# Autodesk Inventor assembly: Assembly_that_isnt_completly broken
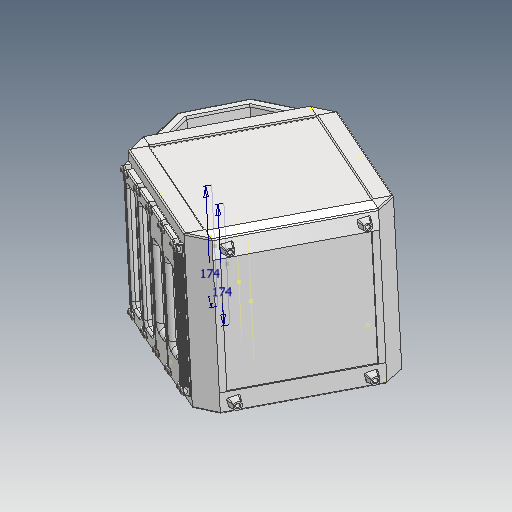
[picture p0: Inventor's stored thumbnail of the model, 512x512]
Saved by Autodesk Inventor 2027 (Build 310192060, 192F)
## iProperties
Created: 2026-07-30
Part Number: Assembly_that_isnt_completly broken
Document SubType Name: Assembly
Designer: prest
Author: prest
## Documents named in this file (14)
- C:\Users\prest\OneDrive\Documents\Projects\Home_Lab_Rack\Assembly_that_isnt_completly broken.iam
- C:\Users\prest\OneDrive\Documents\Projects\Home_Lab_Rack\Strut_Angled.ipt
- C:\Users\prest\OneDrive\Documents\Projects\Home_Lab_Rack\Strut_Horizonal_Bottom.ipt
- C:\Users\prest\OneDrive\Documents\Projects\Home_Lab_Rack\Strut_Horizonal_Top.ipt
- C:\Users\prest\OneDrive\Documents\Projects\Home_Lab_Rack\Strut_Vertical.ipt
- C:\Users\prest\OneDrive\Documents\Projects\Home_Lab_Rack\Panel_Bottom.ipt
- C:\Users\prest\OneDrive\Documents\Projects\Home_Lab_Rack\Panel_Side.ipt
- C:\Users\prest\OneDrive\Documents\Projects\Home_Lab_Rack\MISC\Feet.ipt
- C:\Users\prest\OneDrive\Documents\Projects\Home_Lab_Rack\MISC\Handle.ipt
- C:\Users\prest\OneDrive\Documents\Projects\Home_Lab_Rack\Mounts\router_mount.ipt
- C:\Users\prest\OneDrive\Documents\Projects\Home_Lab_Rack\Mounts\Front_Panel_Breathers.ipt
- C:\Users\prest\OneDrive\Documents\Projects\Home_Lab_Rack\Mounts\mini_PC_mount.ipt
- C:\Users\prest\OneDrive\Documents\Inventor\Content Center Files\R2027\en-US\BS 4168(6)\BS 4168 - M6 x 12(6).ipt
- C:\Users\prest\OneDrive\Documents\Projects\Home_Lab_Rack\Panel_Top.ipt
## Components (62 placed, 13 different names)
1. Strut_Angled:1 — Rigid:5, Rigid:6, Rigid:7, Rotational:32, Rotational:33, Mate:30, Rigid:14
2. Strut_Horizonal_Bottom:1 — Rigid:3, Rigid:5, Rotational:6, Rotational:7
3. Strut_Horizonal_Bottom:2 — Rotational:3, Rotational:4, Rotational:5, Mate:30
4. Strut_Vertical:1 — Rigid:1, Rigid:8, Mate:2, Mate:4, Mate:6, Mate:8, Mate:11, Mate:14, Mate:18, Rigid:11
5. Strut_Angled:2 — Rigid:1, Rigid:3, Rigid:4, Mate:16, Rotational:3
6. Strut_Angled:3 — Rigid:8, Rotational:2, Mate:13, Mate:20, Rotational:36, Rotational:37, Rotational:38, Rotational:39
7. Strut_Vertical:2 — Rigid:4, Mate:1, Mate:3, Mate:5, Mate:7, Mate:9, Mate:10, Mate:12, Mate:15, Mate:17, Rigid:12
8. Strut_Vertical:3 — Rigid:7, Rigid:9
9. Strut_Vertical:4 — Rigid:6
10. Strut_Angled:4 — Rigid:9, Rotational:1, Mate:19, Rotational:34, Rotational:35, Rotational:40, Rotational:41
11. Strut_Horizonal_Top:2 — Rotational:1, Mate:20, Rigid:10
12. Strut_Horizonal_Top:3 — Rotational:2, Mate:19, Mate:21, Mate:22, Rigid:15
13. Feet:1 — Rotational:7
14. router_mount:1 — Mate:1, Mate:2, Mate:3, Rotational:21, Rotational:22, Rotational:24, Rotational:25
15. Front_Panel_Breathers:1 — Mate:13, Mate:14, Mate:15, Rotational:8, Rotational:9
16. mini_PC_mount:1 — Mate:7, Mate:8, Mate:9, Rotational:13, Rotational:15, Rotational:16, Rotational:17
17. router_mount:2 — Mate:4, Mate:5, Mate:6, Rotational:18, Rotational:19, Rotational:20, Rotational:23
18. mini_PC_mount:2 — Mate:10, Mate:11, Mate:12, Rotational:10, Rotational:11, Rotational:12, Rotational:14
19. Front_Panel_Breathers:2 — Mate:16, Mate:17, Mate:18, Rotational:26, Rotational:27
20. Handle:1 — Rigid:10, Rotational:29, Rotational:30
21. Handle:2 — Mate:21, Mate:22, Rotational:28, Rotational:31
22. Feet:2 — Rotational:4
23. Feet:3 — Rotational:5
24. Feet:4 — Rotational:6
25. BS 4168 : Part 6 Hexagon socket countersunk and button head screws - Metric series - Metric M6 x 12:1 — Rotational:32
26. BS 4168 : Part 6 Hexagon socket countersunk and button head screws - Metric series - Metric M6 x 12:2 — Rotational:35
27. BS 4168 : Part 6 Hexagon socket countersunk and button head screws - Metric series - Metric M6 x 12:3 — Rotational:36
28. BS 4168 : Part 6 Hexagon socket countersunk and button head screws - Metric series - Metric M6 x 12:4 — Rotational:37
29. BS 4168 : Part 6 Hexagon socket countersunk and button head screws - Metric series - Metric M6 x 12:5 — Rotational:40
30. BS 4168 : Part 6 Hexagon socket countersunk and button head screws - Metric series - Metric M6 x 12:6 — Rotational:41
31. BS 4168 : Part 6 Hexagon socket countersunk and button head screws - Metric series - Metric M6 x 12:7 — Rotational:9
32. BS 4168 : Part 6 Hexagon socket countersunk and button head screws - Metric series - Metric M6 x 12:8 — Rotational:8
33. BS 4168 : Part 6 Hexagon socket countersunk and button head screws - Metric series - Metric M6 x 12:9 — Rotational:28
34. BS 4168 : Part 6 Hexagon socket countersunk and button head screws - Metric series - Metric M6 x 12:10 — Rotational:34
35. BS 4168 : Part 6 Hexagon socket countersunk and button head screws - Metric series - Metric M6 x 12:11 — Rotational:10
36. BS 4168 : Part 6 Hexagon socket countersunk and button head screws - Metric series - Metric M6 x 12:12 — Rotational:11
37. BS 4168 : Part 6 Hexagon socket countersunk and button head screws - Metric series - Metric M6 x 12:13 — Rotational:12
38. BS 4168 : Part 6 Hexagon socket countersunk and button head screws - Metric series - Metric M6 x 12:14 — Rotational:13
39. BS 4168 : Part 6 Hexagon socket countersunk and button head screws - Metric series - Metric M6 x 12:15 — Rotational:15
40. BS 4168 : Part 6 Hexagon socket countersunk and button head screws - Metric series - Metric M6 x 12:16 — Rotational:14
41. BS 4168 : Part 6 Hexagon socket countersunk and button head screws - Metric series - Metric M6 x 12:17 — Rotational:27
42. BS 4168 : Part 6 Hexagon socket countersunk and button head screws - Metric series - Metric M6 x 12:18 — Rotational:20
43. BS 4168 : Part 6 Hexagon socket countersunk and button head screws - Metric series - Metric M6 x 12:19 — Rotational:19
44. BS 4168 : Part 6 Hexagon socket countersunk and button head screws - Metric series - Metric M6 x 12:20 — Rotational:18
45. BS 4168 : Part 6 Hexagon socket countersunk and button head screws - Metric series - Metric M6 x 12:21 — Rotational:17
46. BS 4168 : Part 6 Hexagon socket countersunk and button head screws - Metric series - Metric M6 x 12:22 — Rotational:16
47. BS 4168 : Part 6 Hexagon socket countersunk and button head screws - Metric series - Metric M6 x 12:23 — Rotational:26
48. BS 4168 : Part 6 Hexagon socket countersunk and button head screws - Metric series - Metric M6 x 12:24 — Rotational:25
49. BS 4168 : Part 6 Hexagon socket countersunk and button head screws - Metric series - Metric M6 x 12:25 — Rotational:24
50. BS 4168 : Part 6 Hexagon socket countersunk and button head screws - Metric series - Metric M6 x 12:26 — Rotational:23
51. BS 4168 : Part 6 Hexagon socket countersunk and button head screws - Metric series - Metric M6 x 12:27 — Rotational:22
52. BS 4168 : Part 6 Hexagon socket countersunk and button head screws - Metric series - Metric M6 x 12:28 — Rotational:21
53. BS 4168 : Part 6 Hexagon socket countersunk and button head screws - Metric series - Metric M6 x 12:29 — Rotational:29
54. BS 4168 : Part 6 Hexagon socket countersunk and button head screws - Metric series - Metric M6 x 12:30 — Rotational:30
55. BS 4168 : Part 6 Hexagon socket countersunk and button head screws - Metric series - Metric M6 x 12:31 — Rotational:31
56. BS 4168 : Part 6 Hexagon socket countersunk and button head screws - Metric series - Metric M6 x 12:32 — Rotational:33
57. BS 4168 : Part 6 Hexagon socket countersunk and button head screws - Metric series - Metric M6 x 12:33 — Rotational:39
58. BS 4168 : Part 6 Hexagon socket countersunk and button head screws - Metric series - Metric M6 x 12:34 — Rotational:38
59. Panel_Side:3 — Rigid:11
60. Panel_Side:4 — Rigid:12
61. Panel_Bottom:1 — Rigid:14
62. Panel_Top:1 — Rigid:15
## Relationships (77: RevoluteJoint 41, Mate 23, WeldJoint 13)
- Rigid:1 [WeldJoint]: Strut_Vertical:1 ↔ Strut_Angled:2
- Rigid:3 [WeldJoint]: Strut_Horizonal_Bottom:1 ↔ Strut_Angled:2
- Rigid:4 [WeldJoint]: Strut_Angled:2 ↔ Strut_Vertical:2
- Rigid:5 [WeldJoint]: Strut_Angled:1 ↔ Strut_Horizonal_Bottom:1
- Rigid:6 [WeldJoint]: Strut_Angled:1 ↔ Strut_Vertical:4
- Rigid:7 [WeldJoint]: Strut_Angled:1 ↔ Strut_Vertical:3
- Rigid:8 [WeldJoint]: Strut_Vertical:1 ↔ Strut_Angled:3
- Rigid:9 [WeldJoint]: Strut_Vertical:3 ↔ Strut_Angled:4
- Rotational:1 [RevoluteJoint]: Strut_Angled:4 ↔ Strut_Horizonal_Top:2
- Rotational:2 [RevoluteJoint]: Strut_Angled:3 ↔ Strut_Horizonal_Top:3
- Mate:1: Strut_Vertical:2 ↔ router_mount:1
- Mate:2: Strut_Vertical:1 ↔ router_mount:1
- Mate:3: Strut_Vertical:2 ↔ router_mount:1
- Mate:4: Strut_Vertical:1 ↔ router_mount:2
- Mate:5: Strut_Vertical:2 ↔ router_mount:2
- Mate:6: Strut_Vertical:1 ↔ router_mount:2
- Mate:7: Strut_Vertical:2 ↔ mini_PC_mount:1
- Mate:8: Strut_Vertical:1 ↔ mini_PC_mount:1
- Mate:9: Strut_Vertical:2 ↔ mini_PC_mount:1
- Mate:10: Strut_Vertical:2 ↔ mini_PC_mount:2
- Mate:11: Strut_Vertical:1 ↔ mini_PC_mount:2
- Mate:12: Strut_Vertical:2 ↔ mini_PC_mount:2
- Mate:13: Strut_Angled:3 ↔ Front_Panel_Breathers:1
- Mate:14: Strut_Vertical:1 ↔ Front_Panel_Breathers:1
- Mate:15: Strut_Vertical:2 ↔ Front_Panel_Breathers:1
- Mate:16: Strut_Angled:2 ↔ Front_Panel_Breathers:2
- Mate:17: Strut_Vertical:2 ↔ Front_Panel_Breathers:2
- Mate:18: Strut_Vertical:1 ↔ Front_Panel_Breathers:2
- Mate:19: Strut_Angled:4 ↔ Strut_Horizonal_Top:3
- Mate:20: Strut_Angled:3 ↔ Strut_Horizonal_Top:2
- Rigid:10 [WeldJoint]: Strut_Horizonal_Top:2 ↔ Handle:1
- Mate:21: Strut_Horizonal_Top:3 ↔ Handle:2
- Mate:22: Strut_Horizonal_Top:3 ↔ Handle:2
- Rotational:3 [RevoluteJoint]: Strut_Horizonal_Bottom:2 ↔ Strut_Angled:2
- Rotational:4 [RevoluteJoint]: Strut_Horizonal_Bottom:2 ↔ Feet:2
- Rotational:5 [RevoluteJoint]: Strut_Horizonal_Bottom:2 ↔ Feet:3
- Rotational:6 [RevoluteJoint]: Strut_Horizonal_Bottom:1 ↔ Feet:4
- Rotational:7 [RevoluteJoint]: Strut_Horizonal_Bottom:1 ↔ Feet:1
- Rotational:8 [RevoluteJoint]: Front_Panel_Breathers:1 ↔ BS 4168 : Part 6 Hexagon socket countersunk and button head screws - Metric series - Metric M6 x 12:8
- Rotational:9 [RevoluteJoint]: Front_Panel_Breathers:1 ↔ BS 4168 : Part 6 Hexagon socket countersunk and button head screws - Metric series - Metric M6 x 12:7
- Rotational:10 [RevoluteJoint]: mini_PC_mount:2 ↔ BS 4168 : Part 6 Hexagon socket countersunk and button head screws - Metric series - Metric M6 x 12:11
- Rotational:11 [RevoluteJoint]: mini_PC_mount:2 ↔ BS 4168 : Part 6 Hexagon socket countersunk and button head screws - Metric series - Metric M6 x 12:12
- Rotational:12 [RevoluteJoint]: mini_PC_mount:2 ↔ BS 4168 : Part 6 Hexagon socket countersunk and button head screws - Metric series - Metric M6 x 12:13
- Rotational:13 [RevoluteJoint]: mini_PC_mount:1 ↔ BS 4168 : Part 6 Hexagon socket countersunk and button head screws - Metric series - Metric M6 x 12:14
- Rotational:14 [RevoluteJoint]: mini_PC_mount:2 ↔ BS 4168 : Part 6 Hexagon socket countersunk and button head screws - Metric series - Metric M6 x 12:16
- Rotational:15 [RevoluteJoint]: mini_PC_mount:1 ↔ BS 4168 : Part 6 Hexagon socket countersunk and button head screws - Metric series - Metric M6 x 12:15
- Rotational:16 [RevoluteJoint]: mini_PC_mount:1 ↔ BS 4168 : Part 6 Hexagon socket countersunk and button head screws - Metric series - Metric M6 x 12:22
- Rotational:17 [RevoluteJoint]: mini_PC_mount:1 ↔ BS 4168 : Part 6 Hexagon socket countersunk and button head screws - Metric series - Metric M6 x 12:21
- Rotational:18 [RevoluteJoint]: router_mount:2 ↔ BS 4168 : Part 6 Hexagon socket countersunk and button head screws - Metric series - Metric M6 x 12:20
- Rotational:19 [RevoluteJoint]: router_mount:2 ↔ BS 4168 : Part 6 Hexagon socket countersunk and button head screws - Metric series - Metric M6 x 12:19
- Rotational:20 [RevoluteJoint]: router_mount:2 ↔ BS 4168 : Part 6 Hexagon socket countersunk and button head screws - Metric series - Metric M6 x 12:18
- Rotational:21 [RevoluteJoint]: router_mount:1 ↔ BS 4168 : Part 6 Hexagon socket countersunk and button head screws - Metric series - Metric M6 x 12:28
- Rotational:22 [RevoluteJoint]: router_mount:1 ↔ BS 4168 : Part 6 Hexagon socket countersunk and button head screws - Metric series - Metric M6 x 12:27
- Rotational:23 [RevoluteJoint]: router_mount:2 ↔ BS 4168 : Part 6 Hexagon socket countersunk and button head screws - Metric series - Metric M6 x 12:26
- Rotational:24 [RevoluteJoint]: router_mount:1 ↔ BS 4168 : Part 6 Hexagon socket countersunk and button head screws - Metric series - Metric M6 x 12:25
- Rotational:25 [RevoluteJoint]: router_mount:1 ↔ BS 4168 : Part 6 Hexagon socket countersunk and button head screws - Metric series - Metric M6 x 12:24
- Rotational:26 [RevoluteJoint]: Front_Panel_Breathers:2 ↔ BS 4168 : Part 6 Hexagon socket countersunk and button head screws - Metric series - Metric M6 x 12:23
- Rotational:27 [RevoluteJoint]: Front_Panel_Breathers:2 ↔ BS 4168 : Part 6 Hexagon socket countersunk and button head screws - Metric series - Metric M6 x 12:17
- Rotational:28 [RevoluteJoint]: Handle:2 ↔ BS 4168 : Part 6 Hexagon socket countersunk and button head screws - Metric series - Metric M6 x 12:9
- Rotational:29 [RevoluteJoint]: Handle:1 ↔ BS 4168 : Part 6 Hexagon socket countersunk and button head screws - Metric series - Metric M6 x 12:29
- Rotational:30 [RevoluteJoint]: Handle:1 ↔ BS 4168 : Part 6 Hexagon socket countersunk and button head screws - Metric series - Metric M6 x 12:30
- Rotational:31 [RevoluteJoint]: Handle:2 ↔ BS 4168 : Part 6 Hexagon socket countersunk and button head screws - Metric series - Metric M6 x 12:31
- Rotational:32 [RevoluteJoint]: Strut_Angled:1 ↔ BS 4168 : Part 6 Hexagon socket countersunk and button head screws - Metric series - Metric M6 x 12:1
- Rotational:33 [RevoluteJoint]: Strut_Angled:1 ↔ BS 4168 : Part 6 Hexagon socket countersunk and button head screws - Metric series - Metric M6 x 12:32
- Rotational:34 [RevoluteJoint]: Strut_Angled:4 ↔ BS 4168 : Part 6 Hexagon socket countersunk and button head screws - Metric series - Metric M6 x 12:10
- Rotational:35 [RevoluteJoint]: Strut_Angled:4 ↔ BS 4168 : Part 6 Hexagon socket countersunk and button head screws - Metric series - Metric M6 x 12:2
- Rotational:36 [RevoluteJoint]: Strut_Angled:3 ↔ BS 4168 : Part 6 Hexagon socket countersunk and button head screws - Metric series - Metric M6 x 12:3
- Rotational:37 [RevoluteJoint]: Strut_Angled:3 ↔ BS 4168 : Part 6 Hexagon socket countersunk and button head screws - Metric series - Metric M6 x 12:4
- Rotational:38 [RevoluteJoint]: Strut_Angled:3 ↔ BS 4168 : Part 6 Hexagon socket countersunk and button head screws - Metric series - Metric M6 x 12:34
- Rotational:39 [RevoluteJoint]: Strut_Angled:3 ↔ BS 4168 : Part 6 Hexagon socket countersunk and button head screws - Metric series - Metric M6 x 12:33
- Rotational:40 [RevoluteJoint]: Strut_Angled:4 ↔ BS 4168 : Part 6 Hexagon socket countersunk and button head screws - Metric series - Metric M6 x 12:5
- Rotational:41 [RevoluteJoint]: Strut_Angled:4 ↔ BS 4168 : Part 6 Hexagon socket countersunk and button head screws - Metric series - Metric M6 x 12:6
- Mate:30: Strut_Angled:1 ↔ Strut_Horizonal_Bottom:2
- Rigid:11 [WeldJoint]: Strut_Vertical:1 ↔ Panel_Side:3
- Rigid:12 [WeldJoint]: Strut_Vertical:2 ↔ Panel_Side:4
- Rigid:14 [WeldJoint]: Strut_Angled:1 ↔ Panel_Bottom:1
- Rigid:15 [WeldJoint]: Strut_Horizonal_Top:3 ↔ Panel_Top:1
